# Autodesk Inventor assembly: 50T nanotube cluster
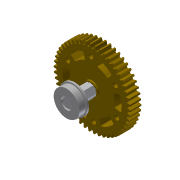
[picture p0: Inventor's stored thumbnail of the model, 180x180]
Saved by Autodesk Inventor 2013 (Build 170138000, 138)
## iProperties
Created: 2013-09-01
Part Number: 50T nanotube cluster
Document SubType Name: Assembly
Designer: Nemo
Author: Nemo
## Documents named in this file (6)
- H:\Nemo\Documents\Robotics\COTS Parts\Gearboxes\Components\50T nanotube cluster.iam
- H:\Nemo\Documents\Robotics\COTS Parts\Gears - VexPro\Gear 20dp 375hex 50T Vex.ipt
- H:\Nemo\Documents\Robotics\COTS Parts\Bearings - VexPro\Flanged Bearing - 0.375in Round ID x 0.875in OD.ipt
- H:\Nemo\Documents\Robotics\COTS Parts\Bearings - AndyMark\Bearing R6zz.ipt
- H:\Nemo\Documents\Robotics\COTS Parts\Gearboxes\Components\VexPro Double Reduction Components\VexBox cluster shaft.ipt
- H:\Nemo\Documents\Robotics\COTS Parts\Gears - VexPro\Gear 20dp 375hex 14T Vex.ipt
## Components (5 placed, 5 different names)
1. Gear 20dp 375hex 50T Vex:1 — Insert:2
2. Flanged Bearing - 0.375in Round ID x 0.875in OD:1
3. Bearing R6zz:1
4. VexBox cluster shaft:1
5. Gear 20dp 375hex 14T Vex:1 — Insert:2
## Relationships (3: Insert 2, Mate 1)
- [Insert]: Bearing R6zz:1 ↔ VexBox cluster shaft:1
- [Mate] (0.254 mm): Gear 20dp 375hex 50T Vex:1 ↔ Bearing R6zz:1
- Insert:2 (0.254 mm): Gear 20dp 375hex 50T Vex:1 ↔ Gear 20dp 375hex 14T Vex:1
